# Autodesk Inventor assembly: Sfu700
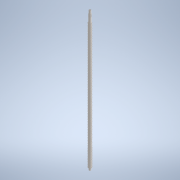
[picture p0: Inventor's stored thumbnail of the model, 180x180]
Saved by Autodesk Inventor 2020.1 (Build 241239000, 239)
## iProperties
Created: 2023-01-06
Part Number: Sfu700
Document SubType Name: Assembly
Designer: KirikDK
Author: KirikDK
## Documents named in this file (3)
- C:\Users\KirikDK\Documents\Stanik1000\Sfu700.iam
- C:\Users\KirikDK\Documents\Stanik1000\SfuObrezki\SFU1605-600start.ipt
- C:\Users\KirikDK\Documents\Stanik1000\SfuObrezki\SFU1605-100end.ipt
## Components (2 placed, 2 different names)
1. SFU1605-600start:1 — Совмещение:1, Совмещение:2
2. SFU1605-100end:1 — Совмещение:1, Совмещение:2
## Relationships (2: Mate 2)
- Совмещение:1 [Mate]: SFU1605-600start:1 ↔ SFU1605-100end:1
- Совмещение:2 [Mate]: SFU1605-600start:1 ↔ SFU1605-100end:1
